# Autodesk Inventor assembly: Ultrasonic sensor assembly
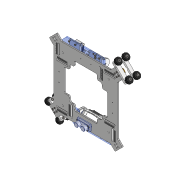
[picture p0: Inventor's stored thumbnail of the model, 180x180]
Saved by Autodesk Inventor 2020 (Build 240168000, 168)
## iProperties
Created: 2020-12-15
Part Number: Ultrasonic sensor assembly
Document SubType Name: Assembly
Designer: ferrerx
Author: ferrerx
## Documents named in this file (10)
- C:\Users\ferrerx\Desktop\Prieto-Godino Lab\Drosophila Larvae Behavioural Device\Device design V3\Inventor Assembly\Ultrasonic sensor assembly.iam
- C:\Users\ferrerx\Desktop\Prieto-Godino Lab\Drosophila Larvae Behavioural Device\Device design V3\Inventor Assembly\Light sources platform.ipt
- C:\Users\ferrerx\Desktop\Prieto-Godino Lab\Drosophila Larvae Behavioural Device\Device design V3\Inventor Assembly\Cart assembly.iam
- C:\Users\ferrerx\Documents\Inventor\Content Center Files\R2020\en-US\AS 1427(05)\AS 1427 - M3 x 25(5) II.ipt
- C:\Users\ferrerx\Desktop\Prieto-Godino Lab\Drosophila Larvae Behavioural Device\Device design V3\Inventor Assembly\Ultrasonic sensor holder.ipt
- C:\Users\ferrerx\Desktop\Prieto-Godino Lab\Drosophila Larvae Behavioural Device\Device design V3\Inventor Assembly\Ultrasonic sensor.ipt
- C:\Users\ferrerx\Documents\Inventor\Content Center Files\R2020\en-US\AS 1427(10)\AS 1427 - M3 x 16(7).ipt
- C:\Users\ferrerx\Documents\Inventor\Content Center Files\R2020\en-US\AS 1427(10)\AS 1427 - M2 x 8(7).ipt
- C:\Users\ferrerx\Documents\Inventor\Content Center Files\R2020\en-US\BS 4183(1)\BS 4183 - M3(1).ipt
- C:\Users\ferrerx\Desktop\Prieto-Godino Lab\Drosophila Larvae Behavioural Device\Device design V3\Inventor Assembly\RGB matrices assembly.iam
## Components (23 placed, 9 different names)
1. Light sources platform:1 — Mate:1, Mate:2, Angle:1, Mate:3, Mate:4, Angle:2, Mate:6, Mate:7, Mate:8, Mate:9, Mate:10, Mate:11, Mate:12, Mate:13, Mate:14, Mate:15, Mate:16, Mate:17, Mate:18, Mate:19, Mate:20, Mate:21, Mate:22, Mate:23, Mate:29, Mate:30, Mate:39, Mate:40, Mate:41, Mate:42, Mate:43, Mate:44
2. Cart assembly:1 [sub-assembly] — Mate:1, Mate:2, Angle:1, Mate:5
3. Cart assembly:2 [sub-assembly] — Mate:3, Mate:4, Angle:2
4. AS 1427 H - Metric M3 x 25:1 — Mate:5, Mate:6
5. AS 1427 H - Metric M3 x 25:2 — Mate:7, Mate:19
6. AS 1427 H - Metric M3 x 25:3 — Mate:9, Mate:20
7. AS 1427 H - Metric M3 x 25:4 — Mate:8, Mate:18
8. AS 1427 H - Metric M3 x 25:5 — Mate:12, Mate:16
9. AS 1427 H - Metric M3 x 25:6 — Mate:10, Mate:17
10. AS 1427 H - Metric M3 x 25:7 — Mate:13, Mate:14
11. AS 1427 H - Metric M3 x 25:8 — Mate:11, Mate:15
12. Ultrasonic sensor holder:1 — Mate:21, Mate:22, Mate:23, Mate:24, Mate:25, Mate:26, Mate:27, Mate:28, Mate:37, Mate:38
13. Ultrasonic sensor:1 — Mate:24, Mate:25, Mate:26, Mate:31, Mate:32, Mate:33, Mate:34
14. AS 1427 (8) - Metric M3 x 16:1 — Mate:27, Mate:30, Mate:36
15. AS 1427 (8) - Metric M3 x 16:2 — Mate:28, Mate:29, Mate:35
16. AS 1427 (8) - Metric M2 x 8:1 — Mate:34
17. AS 1427 (8) - Metric M2 x 8:2 — Mate:31
18. AS 1427 (8) - Metric M2 x 8:3 — Mate:32
19. AS 1427 (8) - Metric M2 x 8:4 — Mate:33
20. BS 4183 - Metric M3:1 — Mate:36, Mate:37
21. BS 4183 - Metric M3:2 — Mate:35, Mate:38
22. RGB matrices assembly:1 [sub-assembly] — Mate:42, Mate:43, Mate:44
23. RGB matrices assembly:2 [sub-assembly] — Mate:39, Mate:40, Mate:41
## Relationships (46: Mate 44, Angle 2)
- Mate:1: Light sources platform:1 ↔ Cart assembly:1
- Mate:2: Light sources platform:1 ↔ Cart assembly:1
- Angle:1 (0 deg): Light sources platform:1 ↔ Cart assembly:1
- Mate:3: Light sources platform:1 ↔ Cart assembly:2
- Mate:4: Light sources platform:1 ↔ Cart assembly:2
- Angle:2 (0 deg): Light sources platform:1 ↔ Cart assembly:2
- Mate:5: Cart assembly:1 ↔ AS 1427 H - Metric M3 x 25:1
- Mate:6: Light sources platform:1 ↔ AS 1427 H - Metric M3 x 25:1
- Mate:7: Light sources platform:1 ↔ AS 1427 H - Metric M3 x 25:2
- Mate:8: Light sources platform:1 ↔ AS 1427 H - Metric M3 x 25:4
- Mate:9: Light sources platform:1 ↔ AS 1427 H - Metric M3 x 25:3
- Mate:10: Light sources platform:1 ↔ AS 1427 H - Metric M3 x 25:6
- Mate:11: Light sources platform:1 ↔ AS 1427 H - Metric M3 x 25:8
- Mate:12: Light sources platform:1 ↔ AS 1427 H - Metric M3 x 25:5
- Mate:13: Light sources platform:1 ↔ AS 1427 H - Metric M3 x 25:7
- Mate:14: Light sources platform:1 ↔ AS 1427 H - Metric M3 x 25:7
- Mate:15: Light sources platform:1 ↔ AS 1427 H - Metric M3 x 25:8
- Mate:16: Light sources platform:1 ↔ AS 1427 H - Metric M3 x 25:5
- Mate:17: Light sources platform:1 ↔ AS 1427 H - Metric M3 x 25:6
- Mate:18: Light sources platform:1 ↔ AS 1427 H - Metric M3 x 25:4
- Mate:19: Light sources platform:1 ↔ AS 1427 H - Metric M3 x 25:2
- Mate:20: Light sources platform:1 ↔ AS 1427 H - Metric M3 x 25:3
- Mate:21: Light sources platform:1 ↔ Ultrasonic sensor holder:1
- Mate:22: Light sources platform:1 ↔ Ultrasonic sensor holder:1
- Mate:23: Light sources platform:1 ↔ Ultrasonic sensor holder:1
- Mate:24: Ultrasonic sensor holder:1 ↔ Ultrasonic sensor:1
- Mate:25: Ultrasonic sensor holder:1 ↔ Ultrasonic sensor:1
- Mate:26: Ultrasonic sensor holder:1 ↔ Ultrasonic sensor:1
- Mate:27: Ultrasonic sensor holder:1 ↔ AS 1427 (8) - Metric M3 x 16:1
- Mate:28: Ultrasonic sensor holder:1 ↔ AS 1427 (8) - Metric M3 x 16:2
- Mate:29: Light sources platform:1 ↔ AS 1427 (8) - Metric M3 x 16:2
- Mate:30: Light sources platform:1 ↔ AS 1427 (8) - Metric M3 x 16:1
- Mate:31: Ultrasonic sensor:1 ↔ AS 1427 (8) - Metric M2 x 8:2
- Mate:32: Ultrasonic sensor:1 ↔ AS 1427 (8) - Metric M2 x 8:3
- Mate:33: Ultrasonic sensor:1 ↔ AS 1427 (8) - Metric M2 x 8:4
- Mate:34: Ultrasonic sensor:1 ↔ AS 1427 (8) - Metric M2 x 8:1
- Mate:35: AS 1427 (8) - Metric M3 x 16:2 ↔ BS 4183 - Metric M3:2
- Mate:36: AS 1427 (8) - Metric M3 x 16:1 ↔ BS 4183 - Metric M3:1
- Mate:37: Ultrasonic sensor holder:1 ↔ BS 4183 - Metric M3:1
- Mate:38: Ultrasonic sensor holder:1 ↔ BS 4183 - Metric M3:2
- Mate:39: Light sources platform:1 ↔ RGB matrices assembly:2
- Mate:40: Light sources platform:1 ↔ RGB matrices assembly:2
- Mate:41: Light sources platform:1 ↔ RGB matrices assembly:2
- Mate:42: Light sources platform:1 ↔ RGB matrices assembly:1
- Mate:43: Light sources platform:1 ↔ RGB matrices assembly:1
- Mate:44: Light sources platform:1 ↔ RGB matrices assembly:1
